# Autodesk Inventor assembly: MG_996R
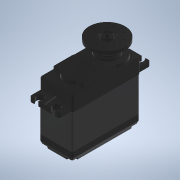
[picture p0: Inventor's stored thumbnail of the model, 180x180]
Saved by Autodesk Inventor 2022 (Build 260153000, 153)
## iProperties
Created: 2016-09-26
Part Number: MG_996R
Document SubType Name: Assembly
Designer: Julian
Author: Julian
## Documents named in this file (6)
- C:\Users\nosal\OneDrive\Pulpit\projekty 3d\Inżynierka\Robot2\silnik\MG_996R.iam
- C:\Users\nosal\OneDrive\Pulpit\projekty 3d\Inżynierka\Robot2\silnik\Base.ipt
- C:\Users\nosal\OneDrive\Pulpit\projekty 3d\Inżynierka\Robot2\silnik\Medio.ipt
- C:\Users\nosal\OneDrive\Pulpit\projekty 3d\Inżynierka\Robot2\silnik\Top.ipt
- C:\Users\nosal\OneDrive\Pulpit\projekty 3d\Inżynierka\Robot2\silnik\Eje.ipt
- C:\Users\nosal\OneDrive\Pulpit\projekty 3d\Inżynierka\Robot2\silnik\Acople circular.ipt
## Components (5 placed, 5 different names)
1. Top:1 — Rígido:2, De rotación:1
2. Medio:1 — Rígido:1, Rígido:2
3. Base:1 — Rígido:1
4. Eje:1 — De rotación:1, De rotación:2
5. Acople circular:1 — De rotación:2
## Relationships (4: WeldJoint 2, RevoluteJoint 2)
- Rígido:1 [WeldJoint]: Medio:1 ↔ Base:1
- Rígido:2 [WeldJoint]: Top:1 ↔ Medio:1
- De rotación:1 [RevoluteJoint]: Top:1 ↔ Eje:1
- De rotación:2 [RevoluteJoint]: Eje:1 ↔ Acople circular:1
